# Autodesk Inventor assembly: Hand_ROCK
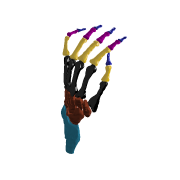
[picture p0: Inventor's stored thumbnail of the model, 180x180]
Saved by Autodesk Inventor 2020 (Build 240168000, 168)
## iProperties
Created: 2021-03-04
Part Number: Hand_ROCK
Document SubType Name: Assembly
Designer: deox
Author: deox
## Documents named in this file (58)
- C:\Users\deox\Documents\Inventor Files\Projeto Punho\Hand_ROCK.iam
- C:\Users\deox\Documents\Inventor Files\Projeto Punho\Bone_1.ipt
- C:\Users\deox\Documents\Inventor Files\Projeto Punho\Radius_v2.ipt
- C:\Users\deox\Documents\Inventor Files\Projeto Punho\Radius_Bone1_Joint.ipt
- C:\Users\deox\Documents\Inventor Files\Projeto Punho\Bone_2.ipt
- C:\Users\deox\Documents\Inventor Files\Projeto Punho\Bone1_2_Joint.ipt
- C:\Users\deox\Documents\Inventor Files\Projeto Punho\Bone_3.ipt
- C:\Users\deox\Documents\Inventor Files\Projeto Punho\Bone3_1_Fix.ipt
- C:\Users\deox\Documents\Inventor Files\Projeto Punho\Bone_4.ipt
- C:\Users\deox\Documents\Inventor Files\Projeto Punho\Bone_4_3_Fix.ipt
- C:\Users\deox\Documents\Inventor Files\Projeto Punho\Ulna.ipt
- C:\Users\deox\Documents\Inventor Files\Projeto Punho\Bone_5.ipt
- C:\Users\deox\Documents\Inventor Files\Projeto Punho\Bone5_4_fix.ipt
- C:\Users\deox\Documents\Inventor Files\Projeto Punho\Bone_6.ipt
- C:\Users\deox\Documents\Inventor Files\Projeto Punho\Bone6_5_Fix.ipt
- C:\Users\deox\Documents\Inventor Files\Projeto Punho\Bone_7.ipt
- C:\Users\deox\Documents\Inventor Files\Projeto Punho\Bone7_1_Fix.ipt
- C:\Users\deox\Documents\Inventor Files\Projeto Punho\Bone_8.ipt
- C:\Users\deox\Documents\Inventor Files\Projeto Punho\Bone8_3_Fix.ipt
- C:\Users\deox\Documents\Inventor Files\Projeto Punho\Bone_9.ipt
- C:\Users\deox\Documents\Inventor Files\Projeto Punho\Bone9_7_Fix.ipt
- C:\Users\deox\Documents\Inventor Files\Projeto Punho\Bone_10.ipt
- C:\Users\deox\Documents\Inventor Files\Projeto Punho\Bone10_8_Fix.ipt
- C:\Users\deox\Documents\Inventor Files\Projeto Punho\Bone_11.ipt
- C:\Users\deox\Documents\Inventor Files\Projeto Punho\Bone11_3_Fix.ipt
- C:\Users\deox\Documents\Inventor Files\Projeto Punho\Bone_12.ipt
- C:\Users\deox\Documents\Inventor Files\Projeto Punho\Bone12_4Fix.ipt
- C:\Users\deox\Documents\Inventor Files\Projeto Punho\Bone_13.ipt
- C:\Users\deox\Documents\Inventor Files\Projeto Punho\Bone13_4_fix.ipt
- C:\Users\deox\Documents\Inventor Files\Projeto Punho\Bone_14.ipt
- C:\Users\deox\Documents\Inventor Files\Projeto Punho\Bone14_9_Fix.ipt
- C:\Users\deox\Documents\Inventor Files\Projeto Punho\Bone_15.ipt
- C:\Users\deox\Documents\Inventor Files\Projeto Punho\Bone15_14_Fix.ipt
- C:\Users\deox\Documents\Inventor Files\Projeto Punho\Bone_16.ipt
- C:\Users\deox\Documents\Inventor Files\Projeto Punho\Bone_17.ipt
- C:\Users\deox\Documents\Inventor Files\Projeto Punho\Bone17_16_Fix.ipt
- C:\Users\deox\Documents\Inventor Files\Projeto Punho\Bone_18.ipt
- C:\Users\deox\Documents\Inventor Files\Projeto Punho\Bone18_17_Fix.ipt
- C:\Users\deox\Documents\Inventor Files\Projeto Punho\Bone_19.ipt
- C:\Users\deox\Documents\Inventor Files\Projeto Punho\Bone19_11_Fix.ipt
- C:\Users\deox\Documents\Inventor Files\Projeto Punho\Bone_20.ipt
- C:\Users\deox\Documents\Inventor Files\Projeto Punho\Bone20_19_Fix.ipt
- C:\Users\deox\Documents\Inventor Files\Projeto Punho\Bone_21.ipt
- C:\Users\deox\Documents\Inventor Files\Projeto Punho\Bone21_20_Fix.ipt
- C:\Users\deox\Documents\Inventor Files\Projeto Punho\Bone_22.ipt
- C:\Users\deox\Documents\Inventor Files\Projeto Punho\Bone22_12_Fix.ipt
- C:\Users\deox\Documents\Inventor Files\Projeto Punho\Bone_23.ipt
- C:\Users\deox\Documents\Inventor Files\Projeto Punho\Bone23_22_Fix.ipt
- C:\Users\deox\Documents\Inventor Files\Projeto Punho\Bone_24.ipt
- C:\Users\deox\Documents\Inventor Files\Projeto Punho\Bone24_23_Fix.ipt
- C:\Users\deox\Documents\Inventor Files\Projeto Punho\Bone_25.ipt
- C:\Users\deox\Documents\Inventor Files\Projeto Punho\Bone25_13_Fix.ipt
- C:\Users\deox\Documents\Inventor Files\Projeto Punho\Bone_26.ipt
- C:\Users\deox\Documents\Inventor Files\Projeto Punho\Bone26_25_Fix.ipt
- C:\Users\deox\Documents\Inventor Files\Projeto Punho\Bone_27.ipt
- C:\Users\deox\Documents\Inventor Files\Projeto Punho\Bone27_26_Fix.ipt
- C:\Users\deox\Documents\Inventor Files\Projeto Punho\Solid2.ipt
- C:\Users\deox\Documents\Inventor Files\Projeto Punho\Solid3.ipt
## Components (57 placed, 57 different names)
1. Bone_1:1 — Mate:1, Mate:5, Mate:6, Mate:7, Mate:8, Mate:15, Mate:16, Mate:17, Mate:39, Mate:40, Mate:41
2. Radius_v2:1 — Mate:2, Mate:3, Mate:4
3. Radius_Bone1_Joint:1 — Mate:1, Mate:2, Mate:3, Mate:4, Mate:5
4. Bone_2:1 — Mate:9, Mate:10, Mate:11
5. Bone1_2_Joint:1 — Mate:6, Mate:7, Mate:8, Mate:9, Mate:10, Mate:11
6. Bone_3:1 — Mate:12, Mate:13, Mate:14, Mate:21, Mate:22, Mate:23, Mate:45, Mate:46, Mate:47, Mate:61, Mate:62, Mate:63
7. Bone3_1_Fix:1 — Mate:12, Mate:13, Mate:14, Mate:15, Mate:16, Mate:17
8. Bone_4:1 — Mate:18, Mate:19, Mate:20, Mate:27, Mate:28, Mate:29, Mate:66, Mate:67, Mate:70, Mate:71
9. Bone_4_3_Fix:1 — Mate:18, Mate:19, Mate:20, Mate:21, Mate:22, Mate:23
10. Ulna:1
11. Bone_5:1 — Mate:24, Mate:25, Mate:26, Mate:33, Mate:34, Mate:35
12. Bone5_4_fix:1 — Mate:24, Mate:25, Mate:26, Mate:27, Mate:28, Mate:29
13. Bone_6:1 — Mate:30, Mate:31, Mate:32
14. Bone6_5_Fix:1 — Mate:30, Mate:31, Mate:32, Mate:33, Mate:34, Mate:35
15. Bone_7:1 — Mate:36, Mate:37, Mate:38, Mate:50, Mate:51
16. Bone7_1_Fix:1 — Mate:36, Mate:37, Mate:38, Mate:39, Mate:40, Mate:41
17. Bone_8:1 — Mate:42, Mate:43, Mate:44, Mate:55, Mate:56, Mate:57
18. Bone8_3_Fix:1 — Mate:42, Mate:43, Mate:44, Mate:45, Mate:46, Mate:47
19. Bone_9:1 — Mate:48, Mate:49, Mate:74, Mate:75, Mate:76
20. Bone9_7_Fix:1 — Mate:48, Mate:49, Mate:50, Mate:51
21. Bone_10:1 — Mate:52, Mate:53, Mate:54, Angle:4, Mate:145, Mate:146, Mate:149
22. Bone10_8_Fix:1 — Mate:52, Mate:53, Mate:54, Mate:55, Mate:56, Mate:57
23. Bone_11:1 — Mate:58, Mate:59, Mate:60, Angle:2, Angle:3, Mate:99, Mate:100, Mate:101
24. Bone11_3_Fix:1 — Mate:58, Mate:59, Mate:60, Mate:61, Mate:62, Mate:63
25. Bone_12:1 — Mate:64, Mate:65, Angle:2, Mate:114, Mate:115, Mate:118
26. Bone12_4Fix:1 — Mate:64, Mate:65, Mate:66, Mate:67
27. Bone_13:1 — Mate:68, Mate:69, Angle:3, Mate:131, Mate:132, Mate:133
28. Bone13_4_fix:1 — Mate:68, Mate:69, Mate:70, Mate:71
29. Bone_14:1 — Mate:72, Mate:73, Angle:4, Mate:79, Mate:80, Mate:81
30. Bone14_9_Fix:1 — Mate:72, Mate:73, Mate:74, Mate:75, Mate:76
31. Bone_15:1 — Mate:77, Mate:78
32. Bone15_14_Fix:1 — Mate:77, Mate:78, Mate:79, Mate:80, Mate:81
33. Bone_16:1 — Mate:89, Mate:90, Mate:91, Mate:147, Mate:148
34. Bone_17:1 — Mate:87, Mate:88, Mate:94, Mate:95, Mate:96
35. Bone17_16_Fix:1 — Mate:87, Mate:88, Mate:89, Mate:90, Mate:91
36. Bone_18:1 — Mate:92, Mate:93
37. Bone18_17_Fix:1 — Mate:92, Mate:93, Mate:94, Mate:95, Mate:96
38. Bone_19:1 — Mate:97, Mate:98, Mate:104, Mate:105, Mate:106
39. Bone19_11_Fix:1 — Mate:97, Mate:98, Mate:99, Mate:100, Mate:101
40. Bone_20:1 — Mate:102, Mate:103, Mate:109, Mate:110, Mate:111
41. Bone20_19_Fix:1 — Mate:102, Mate:103, Mate:104, Mate:105, Mate:106
42. Bone_21:1 — Mate:107, Mate:108
43. Bone21_20_Fix:1 — Mate:107, Mate:108, Mate:109, Mate:110, Mate:111
44. Bone_22:1 — Mate:113, Mate:116, Mate:117, Mate:121, Mate:122, Mate:123
45. Bone22_12_Fix:1 — Mate:113, Mate:114, Mate:115, Mate:116, Mate:117, Mate:118
46. Bone_23:1 — Mate:119, Mate:120, Mate:126, Mate:127, Mate:128
47. Bone23_22_Fix:1 — Mate:119, Mate:120, Mate:121, Mate:122, Mate:123
48. Bone_24:1 — Mate:124, Mate:125
49. Bone24_23_Fix:1 — Mate:124, Mate:125, Mate:126, Mate:127, Mate:128
50. Bone_25:1 — Mate:129, Mate:130, Mate:136, Mate:137, Mate:138
51. Bone25_13_Fix:1 — Mate:129, Mate:130, Mate:131, Mate:132, Mate:133
52. Bone_26:1 — Mate:134, Mate:135, Mate:141, Mate:142, Mate:143
53. Bone26_25_Fix:1 — Mate:134, Mate:135, Mate:136, Mate:137, Mate:138
54. Bone_27:1 — Mate:139, Mate:140
55. Bone27_26_Fix:1 — Mate:139, Mate:140, Mate:141, Mate:142, Mate:143
56. Solid2:1 — Mate:144, Flush:1, Angle:5, Mate:147, Mate:148
57. Solid3:1 — Mate:144, Flush:1, Angle:5, Mate:145, Mate:146, Mate:149
## Relationships (148: Mate 143, Angle 4, Flush 1)
- Mate:1: Bone_1:1 ↔ Radius_Bone1_Joint:1
- Mate:2: Radius_v2:1 ↔ Radius_Bone1_Joint:1
- Mate:3: Radius_v2:1 ↔ Radius_Bone1_Joint:1
- Mate:4: Radius_v2:1 ↔ Radius_Bone1_Joint:1
- Mate:5: Bone_1:1 ↔ Radius_Bone1_Joint:1
- Mate:6: Bone_1:1 ↔ Bone1_2_Joint:1
- Mate:7: Bone_1:1 ↔ Bone1_2_Joint:1
- Mate:8: Bone_1:1 ↔ Bone1_2_Joint:1
- Mate:9: Bone_2:1 ↔ Bone1_2_Joint:1
- Mate:10: Bone_2:1 ↔ Bone1_2_Joint:1
- Mate:11: Bone_2:1 ↔ Bone1_2_Joint:1
- Mate:12: Bone_3:1 ↔ Bone3_1_Fix:1
- Mate:13: Bone_3:1 ↔ Bone3_1_Fix:1
- Mate:14: Bone_3:1 ↔ Bone3_1_Fix:1
- Mate:15: Bone_1:1 ↔ Bone3_1_Fix:1
- Mate:16: Bone_1:1 ↔ Bone3_1_Fix:1
- Mate:17: Bone_1:1 ↔ Bone3_1_Fix:1
- Mate:18: Bone_4:1 ↔ Bone_4_3_Fix:1
- Mate:19: Bone_4:1 ↔ Bone_4_3_Fix:1
- Mate:20: Bone_4:1 ↔ Bone_4_3_Fix:1
- Mate:21: Bone_3:1 ↔ Bone_4_3_Fix:1
- Mate:22: Bone_3:1 ↔ Bone_4_3_Fix:1
- Mate:23: Bone_3:1 ↔ Bone_4_3_Fix:1
- Mate:24: Bone_5:1 ↔ Bone5_4_fix:1
- Mate:25: Bone_5:1 ↔ Bone5_4_fix:1
- Mate:26: Bone_5:1 ↔ Bone5_4_fix:1
- Mate:27: Bone_4:1 ↔ Bone5_4_fix:1
- Mate:28: Bone_4:1 ↔ Bone5_4_fix:1
- Mate:29: Bone_4:1 ↔ Bone5_4_fix:1
- Mate:30: Bone_6:1 ↔ Bone6_5_Fix:1
- Mate:31: Bone_6:1 ↔ Bone6_5_Fix:1
- Mate:32: Bone_6:1 ↔ Bone6_5_Fix:1
- Mate:33: Bone_5:1 ↔ Bone6_5_Fix:1
- Mate:34: Bone_5:1 ↔ Bone6_5_Fix:1
- Mate:35: Bone_5:1 ↔ Bone6_5_Fix:1
- Mate:36: Bone_7:1 ↔ Bone7_1_Fix:1
- Mate:37: Bone_7:1 ↔ Bone7_1_Fix:1
- Mate:38: Bone_7:1 ↔ Bone7_1_Fix:1
- Mate:39: Bone_1:1 ↔ Bone7_1_Fix:1
- Mate:40: Bone_1:1 ↔ Bone7_1_Fix:1
- Mate:41: Bone_1:1 ↔ Bone7_1_Fix:1
- Mate:42: Bone_8:1 ↔ Bone8_3_Fix:1
- Mate:43: Bone_8:1 ↔ Bone8_3_Fix:1
- Mate:44: Bone_8:1 ↔ Bone8_3_Fix:1
- Mate:45: Bone_3:1 ↔ Bone8_3_Fix:1
- Mate:46: Bone_3:1 ↔ Bone8_3_Fix:1
- Mate:47: Bone_3:1 ↔ Bone8_3_Fix:1
- Mate:48: Bone_9:1 ↔ Bone9_7_Fix:1
- Mate:49: Bone_9:1 ↔ Bone9_7_Fix:1
- Mate:50: Bone_7:1 ↔ Bone9_7_Fix:1
- Mate:51: Bone_7:1 ↔ Bone9_7_Fix:1
- Mate:52: Bone_10:1 ↔ Bone10_8_Fix:1
- Mate:53: Bone_10:1 ↔ Bone10_8_Fix:1
- Mate:54: Bone_10:1 ↔ Bone10_8_Fix:1
- Mate:55: Bone_8:1 ↔ Bone10_8_Fix:1
- Mate:56: Bone_8:1 ↔ Bone10_8_Fix:1
- Mate:57: Bone_8:1 ↔ Bone10_8_Fix:1
- Mate:58: Bone_11:1 ↔ Bone11_3_Fix:1
- Mate:59: Bone_11:1 ↔ Bone11_3_Fix:1
- Mate:60: Bone_11:1 ↔ Bone11_3_Fix:1
- Mate:61: Bone_3:1 ↔ Bone11_3_Fix:1
- Mate:62: Bone_3:1 ↔ Bone11_3_Fix:1
- Mate:63: Bone_3:1 ↔ Bone11_3_Fix:1
- Mate:64: Bone_12:1 ↔ Bone12_4Fix:1
- Mate:65: Bone_12:1 ↔ Bone12_4Fix:1
- Mate:66: Bone_4:1 ↔ Bone12_4Fix:1
- Mate:67: Bone_4:1 ↔ Bone12_4Fix:1
- Angle:2 (0 deg): Bone_11:1 ↔ Bone_12:1
- Mate:68: Bone_13:1 ↔ Bone13_4_fix:1
- Mate:69: Bone_13:1 ↔ Bone13_4_fix:1
- Mate:70: Bone_4:1 ↔ Bone13_4_fix:1
- Mate:71: Bone_4:1 ↔ Bone13_4_fix:1
- Angle:3 (0 deg): Bone_11:1 ↔ Bone_13:1
- Mate:72: Bone_14:1 ↔ Bone14_9_Fix:1
- Mate:73: Bone_14:1 ↔ Bone14_9_Fix:1
- Mate:74: Bone_9:1 ↔ Bone14_9_Fix:1
- Mate:75: Bone_9:1 ↔ Bone14_9_Fix:1
- Mate:76: Bone_9:1 ↔ Bone14_9_Fix:1
- Angle:4 (0 deg): Bone_10:1 ↔ Bone_14:1
- Mate:77: Bone_15:1 ↔ Bone15_14_Fix:1
- Mate:78: Bone_15:1 ↔ Bone15_14_Fix:1
- Mate:79: Bone_14:1 ↔ Bone15_14_Fix:1
- Mate:80: Bone_14:1 ↔ Bone15_14_Fix:1
- Mate:81: Bone_14:1 ↔ Bone15_14_Fix:1
- Mate:87: Bone_17:1 ↔ Bone17_16_Fix:1
- Mate:88: Bone_17:1 ↔ Bone17_16_Fix:1
- Mate:89: Bone_16:1 ↔ Bone17_16_Fix:1
- Mate:90: Bone_16:1 ↔ Bone17_16_Fix:1
- Mate:91: Bone_16:1 ↔ Bone17_16_Fix:1
- Mate:92: Bone_18:1 ↔ Bone18_17_Fix:1
- Mate:93: Bone_18:1 ↔ Bone18_17_Fix:1
- Mate:94: Bone_17:1 ↔ Bone18_17_Fix:1
- Mate:95: Bone_17:1 ↔ Bone18_17_Fix:1
- Mate:96: Bone_17:1 ↔ Bone18_17_Fix:1
- Mate:97: Bone_19:1 ↔ Bone19_11_Fix:1
- Mate:98: Bone_19:1 ↔ Bone19_11_Fix:1
- Mate:99: Bone_11:1 ↔ Bone19_11_Fix:1
- Mate:100: Bone_11:1 ↔ Bone19_11_Fix:1
- Mate:101: Bone_11:1 ↔ Bone19_11_Fix:1
- Mate:102: Bone_20:1 ↔ Bone20_19_Fix:1
- Mate:103: Bone_20:1 ↔ Bone20_19_Fix:1
- Mate:104: Bone_19:1 ↔ Bone20_19_Fix:1
- Mate:105: Bone_19:1 ↔ Bone20_19_Fix:1
- Mate:106: Bone_19:1 ↔ Bone20_19_Fix:1
- Mate:107: Bone_21:1 ↔ Bone21_20_Fix:1
- Mate:108: Bone_21:1 ↔ Bone21_20_Fix:1
- Mate:109: Bone_20:1 ↔ Bone21_20_Fix:1
- Mate:110: Bone_20:1 ↔ Bone21_20_Fix:1
- Mate:111: Bone_20:1 ↔ Bone21_20_Fix:1
- Mate:113: Bone_22:1 ↔ Bone22_12_Fix:1
- Mate:114: Bone_12:1 ↔ Bone22_12_Fix:1
- Mate:115: Bone_12:1 ↔ Bone22_12_Fix:1
- Mate:116: Bone_22:1 ↔ Bone22_12_Fix:1
- Mate:117: Bone_22:1 ↔ Bone22_12_Fix:1
- Mate:118: Bone_12:1 ↔ Bone22_12_Fix:1
- Mate:119: Bone_23:1 ↔ Bone23_22_Fix:1
- Mate:120: Bone_23:1 ↔ Bone23_22_Fix:1
- Mate:121: Bone_22:1 ↔ Bone23_22_Fix:1
- Mate:122: Bone_22:1 ↔ Bone23_22_Fix:1
- Mate:123: Bone_22:1 ↔ Bone23_22_Fix:1
- Mate:124: Bone_24:1 ↔ Bone24_23_Fix:1
- Mate:125: Bone_24:1 ↔ Bone24_23_Fix:1
- Mate:126: Bone_23:1 ↔ Bone24_23_Fix:1
- Mate:127: Bone_23:1 ↔ Bone24_23_Fix:1
- Mate:128: Bone_23:1 ↔ Bone24_23_Fix:1
- Mate:129: Bone_25:1 ↔ Bone25_13_Fix:1
- Mate:130: Bone_25:1 ↔ Bone25_13_Fix:1
- Mate:131: Bone_13:1 ↔ Bone25_13_Fix:1
- Mate:132: Bone_13:1 ↔ Bone25_13_Fix:1
- Mate:133: Bone_13:1 ↔ Bone25_13_Fix:1
- Mate:134: Bone_26:1 ↔ Bone26_25_Fix:1
- Mate:135: Bone_26:1 ↔ Bone26_25_Fix:1
- Mate:136: Bone_25:1 ↔ Bone26_25_Fix:1
- Mate:137: Bone_25:1 ↔ Bone26_25_Fix:1
- Mate:138: Bone_25:1 ↔ Bone26_25_Fix:1
- Mate:139: Bone_27:1 ↔ Bone27_26_Fix:1
- Mate:140: Bone_27:1 ↔ Bone27_26_Fix:1
- Mate:141: Bone_26:1 ↔ Bone27_26_Fix:1
- Mate:142: Bone_26:1 ↔ Bone27_26_Fix:1
- Mate:143: Bone_26:1 ↔ Bone27_26_Fix:1
- Mate:144: Solid2:1 ↔ Solid3:1
- Flush:1: Solid2:1 ↔ Solid3:1
- Angle:5 (0 deg): Solid2:1 ↔ Solid3:1
- Mate:145: Bone_10:1 ↔ Solid3:1
- Mate:146: Bone_10:1 ↔ Solid3:1
- Mate:147: Bone_16:1 ↔ Solid2:1
- Mate:148: Bone_16:1 ↔ Solid2:1
- Mate:149: Bone_10:1 ↔ Solid3:1
